# Autodesk Inventor assembly: ODrive Pro Assembly
(part 2 of 2)
- C:\work\openworkout\digital_weight_device\cad\v5\odrive\ODrive Pro Assembly\Leader_6_1.ipt
- C:\work\openworkout\digital_weight_device\cad\v5\odrive\ODrive Pro Assembly\Extruded_4_6.ipt
- C:\work\openworkout\digital_weight_device\cad\v5\odrive\ODrive Pro Assembly\Open CASCADE STEP translator 6.8 2.1.1_2_1.ipt
- C:\work\openworkout\digital_weight_device\cad\v5\odrive\ODrive Pro Assembly\Extruded_4_7.ipt
- C:\work\openworkout\digital_weight_device\cad\v5\odrive\ODrive Pro Assembly\Cylinder_6_2.ipt
- C:\work\openworkout\digital_weight_device\cad\v5\odrive\ODrive Pro Assembly\Lead_2.ipt
- C:\work\openworkout\digital_weight_device\cad\v5\odrive\ODrive Pro Assembly\RES 0603 (1608 metric)_8.ipt
- C:\work\openworkout\digital_weight_device\cad\v5\odrive\ODrive Pro Assembly\Open CASCADE STEP translator 6.8 1.2.1_2_1.ipt
- C:\work\openworkout\digital_weight_device\cad\v5\odrive\ODrive Pro Assembly\Extruded_21_4.ipt
- C:\work\openworkout\digital_weight_device\cad\v5\odrive\ODrive Pro Assembly\Extruded_58_1.ipt
- C:\work\openworkout\digital_weight_device\cad\v5\odrive\ODrive Pro Assembly\Extruded_64_1.ipt
- C:\work\openworkout\digital_weight_device\cad\v5\odrive\ODrive Pro Assembly\Extruded_38_1.ipt
- C:\work\openworkout\digital_weight_device\cad\v5\odrive\ODrive Pro Assembly\Extruded_39_3.ipt
- C:\work\openworkout\digital_weight_device\cad\v5\odrive\ODrive Pro Assembly\Thermal_Shape.ipt
- C:\work\openworkout\digital_weight_device\cad\v5\odrive\ODrive Pro Assembly\FDMS86300DC rev A.ipt
- C:\work\openworkout\digital_weight_device\cad\v5\odrive\ODrive Pro Assembly\________10 SIZE CODE G_7.ipt
- C:\work\openworkout\digital_weight_device\cad\v5\odrive\ODrive Pro Assembly\Extruded_27_1.ipt
- C:\work\openworkout\digital_weight_device\cad\v5\odrive\ODrive Pro Assembly\Extruded_28_5.ipt
- C:\work\openworkout\digital_weight_device\cad\v5\odrive\ODrive Pro Assembly\Mark_3_4.ipt
- C:\work\openworkout\digital_weight_device\cad\v5\odrive\ODrive Pro Assembly\Open CASCADE STEP translator 6.8 23.2.1_4_2.ipt
- C:\work\openworkout\digital_weight_device\cad\v5\odrive\ODrive Pro Assembly\Extruded_26_1.ipt
- C:\work\openworkout\digital_weight_device\cad\v5\odrive\ODrive Pro Assembly\Extruded_14_9.ipt
- C:\work\openworkout\digital_weight_device\cad\v5\odrive\ODrive Pro Assembly\______10 SIZE CODE G_1.ipt
- C:\work\openworkout\digital_weight_device\cad\v5\odrive\ODrive Pro Assembly\Leader_26.ipt
- C:\work\openworkout\digital_weight_device\cad\v5\odrive\ODrive Pro Assembly\Extruded_66.ipt
- C:\work\openworkout\digital_weight_device\cad\v5\odrive\ODrive Pro Assembly\Mark_1_4.ipt
- C:\work\openworkout\digital_weight_device\cad\v5\odrive\ODrive Pro Assembly\Mark_1_5.ipt
- C:\work\openworkout\digital_weight_device\cad\v5\odrive\ODrive Pro Assembly\Extruded_8_7.ipt
- C:\work\openworkout\digital_weight_device\cad\v5\odrive\ODrive Pro Assembly\Extruded_45_1.ipt
- C:\work\openworkout\digital_weight_device\cad\v5\odrive\ODrive Pro Assembly\Extruded_27_2.ipt
- C:\work\openworkout\digital_weight_device\cad\v5\odrive\ODrive Pro Assembly\Extruded_25_4.ipt
- C:\work\openworkout\digital_weight_device\cad\v5\odrive\ODrive Pro Assembly\FDMS86300DC rev A_11.ipt
- C:\work\openworkout\digital_weight_device\cad\v5\odrive\ODrive Pro Assembly\Extruded_16_5.ipt
- C:\work\openworkout\digital_weight_device\cad\v5\odrive\ODrive Pro Assembly\Extruded_51_1.ipt
- C:\work\openworkout\digital_weight_device\cad\v5\odrive\ODrive Pro Assembly\Open CASCADE STEP translator 6.8 23.2.1_7_1.ipt
- C:\work\openworkout\digital_weight_device\cad\v5\odrive\ODrive Pro Assembly\Open CASCADE STEP translator 6.8 1.2.1_5_1.ipt
- C:\work\openworkout\digital_weight_device\cad\v5\odrive\ODrive Pro Assembly\Cylinder_4_1.ipt
- C:\work\openworkout\digital_weight_device\cad\v5\odrive\ODrive Pro Assembly\Open CASCADE STEP translator 6.8 1.2.1_6.ipt
- C:\work\openworkout\digital_weight_device\cad\v5\odrive\ODrive Pro Assembly\RES 0603 (1608 metric)_19.ipt
- C:\work\openworkout\digital_weight_device\cad\v5\odrive\ODrive Pro Assembly\Extruded_5_10.ipt
- C:\work\openworkout\digital_weight_device\cad\v5\odrive\ODrive Pro Assembly\Extruded_21_5.ipt
- C:\work\openworkout\digital_weight_device\cad\v5\odrive\ODrive Pro Assembly\Mid_Body_6_1.ipt
- C:\work\openworkout\digital_weight_device\cad\v5\odrive\ODrive Pro Assembly\Extruded_23_4.ipt
- C:\work\openworkout\digital_weight_device\cad\v5\odrive\ODrive Pro Assembly\Cylinder_10_2.ipt
- C:\work\openworkout\digital_weight_device\cad\v5\odrive\ODrive Pro Assembly\Extruded_16_6.ipt
- C:\work\openworkout\digital_weight_device\cad\v5\odrive\ODrive Pro Assembly\Extruded_31_3.ipt
- C:\work\openworkout\digital_weight_device\cad\v5\odrive\ODrive Pro Assembly\Leader_4_2.ipt
- C:\work\openworkout\digital_weight_device\cad\v5\odrive\ODrive Pro Assembly\Leader_1_2.ipt
- C:\work\openworkout\digital_weight_device\cad\v5\odrive\ODrive Pro Assembly\Leader_12.ipt
- C:\work\openworkout\digital_weight_device\cad\v5\odrive\ODrive Pro Assembly\Leader_8.ipt
- C:\work\openworkout\digital_weight_device\cad\v5\odrive\ODrive Pro Assembly\Extruded_20_4.ipt
- C:\work\openworkout\digital_weight_device\cad\v5\odrive\ODrive Pro Assembly\Extruded_18_4.ipt
- C:\work\openworkout\digital_weight_device\cad\v5\odrive\ODrive Pro Assembly\RES 0603 (1608 metric)_4.ipt
- C:\work\openworkout\digital_weight_device\cad\v5\odrive\ODrive Pro Assembly\Open CASCADE STEP translator 6.8 2.1.1_7.ipt
- C:\work\openworkout\digital_weight_device\cad\v5\odrive\ODrive Pro Assembly\Extruded_4_8.ipt
- C:\work\openworkout\digital_weight_device\cad\v5\odrive\ODrive Pro Assembly\Extruded_8_8.ipt
- C:\work\openworkout\digital_weight_device\cad\v5\odrive\ODrive Pro Assembly\Cylinder_14.ipt
- C:\work\openworkout\digital_weight_device\cad\v5\odrive\ODrive Pro Assembly\Extruded_17_2.ipt
- C:\work\openworkout\digital_weight_device\cad\v5\odrive\ODrive Pro Assembly\Extruded_14_10.ipt
- C:\work\openworkout\digital_weight_device\cad\v5\odrive\ODrive Pro Assembly\Extruded_9_8.ipt
- C:\work\openworkout\digital_weight_device\cad\v5\odrive\ODrive Pro Assembly\Extruded_4_9.ipt
- C:\work\openworkout\digital_weight_device\cad\v5\odrive\ODrive Pro Assembly\Open CASCADE STEP translator 6.8 43.4.1_8.ipt
- C:\work\openworkout\digital_weight_device\cad\v5\odrive\ODrive Pro Assembly\Open CASCADE STEP translator 6.8 43.4.1_4.ipt
- C:\work\openworkout\digital_weight_device\cad\v5\odrive\ODrive Pro Assembly\Open CASCADE STEP translator 6.8 1.1.ipt
- C:\work\openworkout\digital_weight_device\cad\v5\odrive\ODrive Pro Assembly\Extruded_2_9.ipt
- C:\work\openworkout\digital_weight_device\cad\v5\odrive\ODrive Pro Assembly\Extruded_1_11.ipt
- C:\work\openworkout\digital_weight_device\cad\v5\odrive\ODrive Pro Assembly\Extruded_1_12.ipt
- C:\work\openworkout\digital_weight_device\cad\v5\odrive\ODrive Pro Assembly\Cylinder_10_3.ipt
- C:\work\openworkout\digital_weight_device\cad\v5\odrive\ODrive Pro Assembly\Extruded_3_11.ipt
- C:\work\openworkout\digital_weight_device\cad\v5\odrive\ODrive Pro Assembly\Extruded_1_13.ipt
- C:\work\openworkout\digital_weight_device\cad\v5\odrive\ODrive Pro Assembly\Open CASCADE STEP translator 6.8 2.2.1_3.ipt
- C:\work\openworkout\digital_weight_device\cad\v5\odrive\ODrive Pro Assembly\Open CASCADE STEP translator 6.8 19.1.2.ipt
- C:\work\openworkout\digital_weight_device\cad\v5\odrive\ODrive Pro Assembly\Extruded_2_10.ipt
- C:\work\openworkout\digital_weight_device\cad\v5\odrive\ODrive Pro Assembly\Extruded_67.ipt
- C:\work\openworkout\digital_weight_device\cad\v5\odrive\ODrive Pro Assembly\Extruded_21_6.ipt
- C:\work\openworkout\digital_weight_device\cad\v5\odrive\ODrive Pro Assembly\Extruded_15_8.ipt
- C:\work\openworkout\digital_weight_device\cad\v5\odrive\ODrive Pro Assembly\Leader_3_1.ipt
- C:\work\openworkout\digital_weight_device\cad\v5\odrive\ODrive Pro Assembly\Extruded_56_1.ipt
- C:\work\openworkout\digital_weight_device\cad\v5\odrive\ODrive Pro Assembly\Open CASCADE STEP translator 6.8 26.4.1_4.ipt
- C:\work\openworkout\digital_weight_device\cad\v5\odrive\ODrive Pro Assembly\Mark_9.ipt
- C:\work\openworkout\digital_weight_device\cad\v5\odrive\ODrive Pro Assembly\FDMS86300DC rev A_9.ipt
- C:\work\openworkout\digital_weight_device\cad\v5\odrive\ODrive Pro Assembly\FDMS86300DC rev A_5.ipt
- C:\work\openworkout\digital_weight_device\cad\v5\odrive\ODrive Pro Assembly\Extruded_45_2.ipt
- C:\work\openworkout\digital_weight_device\cad\v5\odrive\ODrive Pro Assembly\Open CASCADE STEP translator 6.8 1.2.1_3_1.ipt
- C:\work\openworkout\digital_weight_device\cad\v5\odrive\ODrive Pro Assembly\Open CASCADE STEP translator 6.8 1.2.1_1_1.ipt
- C:\work\openworkout\digital_weight_device\cad\v5\odrive\ODrive Pro Assembly\Extruded_27_3.ipt
- C:\work\openworkout\digital_weight_device\cad\v5\odrive\ODrive Pro Assembly\Extruded_30_4.ipt
- C:\work\openworkout\digital_weight_device\cad\v5\odrive\ODrive Pro Assembly\Open CASCADE STEP translator 6.8 23.2.1_14.ipt
- C:\work\openworkout\digital_weight_device\cad\v5\odrive\ODrive Pro Assembly\Extruded_17_3.ipt
- C:\work\openworkout\digital_weight_device\cad\v5\odrive\ODrive Pro Assembly\Extruded_16_7.ipt
- C:\work\openworkout\digital_weight_device\cad\v5\odrive\ODrive Pro Assembly\Cylinder_5_1.ipt
- C:\work\openworkout\digital_weight_device\cad\v5\odrive\ODrive Pro Assembly\Extruded_37_2.ipt
- C:\work\openworkout\digital_weight_device\cad\v5\odrive\ODrive Pro Assembly\Extruded_32_4.ipt
- C:\work\openworkout\digital_weight_device\cad\v5\odrive\ODrive Pro Assembly\Extruded_13_8.ipt
- C:\work\openworkout\digital_weight_device\cad\v5\odrive\ODrive Pro Assembly\Mark_2_4.ipt
- C:\work\openworkout\digital_weight_device\cad\v5\odrive\ODrive Pro Assembly\Extruded_18_5.ipt
- C:\work\openworkout\digital_weight_device\cad\v5\odrive\ODrive Pro Assembly\Extruded_38_2.ipt
- C:\work\openworkout\digital_weight_device\cad\v5\odrive\ODrive Pro Assembly\Extruded_11_7.ipt
- C:\work\openworkout\digital_weight_device\cad\v5\odrive\ODrive Pro Assembly\Extruded_4_10.ipt
- C:\work\openworkout\digital_weight_device\cad\v5\odrive\ODrive Pro Assembly\_______10x9.5L SIDE CODE G.ipt
- C:\work\openworkout\digital_weight_device\cad\v5\odrive\ODrive Pro Assembly\Extruded_17_4.ipt
- C:\work\openworkout\digital_weight_device\cad\v5\odrive\ODrive Pro Assembly\________10 SIZE CODE G_4.ipt
- C:\work\openworkout\digital_weight_device\cad\v5\odrive\ODrive Pro Assembly\_______10x9.5L SIDE CODE G_2.ipt
- C:\work\openworkout\digital_weight_device\cad\v5\odrive\ODrive Pro Assembly\Extruded_6_10.ipt
- C:\work\openworkout\digital_weight_device\cad\v5\odrive\ODrive Pro Assembly\Open CASCADE STEP translator 6.8 23.2.1_7_2.ipt
- C:\work\openworkout\digital_weight_device\cad\v5\odrive\ODrive Pro Assembly\Extruded_25_5.ipt
- C:\work\openworkout\digital_weight_device\cad\v5\odrive\ODrive Pro Assembly\Extruded_68.ipt
- C:\work\openworkout\digital_weight_device\cad\v5\odrive\ODrive Pro Assembly\LED 0603 APT1608 GREEN.ipt
- C:\work\openworkout\digital_weight_device\cad\v5\odrive\ODrive Pro Assembly\Extruded_2_11.ipt
- C:\work\openworkout\digital_weight_device\cad\v5\odrive\ODrive Pro Assembly\Mid_Body_10.ipt
- C:\work\openworkout\digital_weight_device\cad\v5\odrive\ODrive Pro Assembly\Mid_Body_1_4.ipt
- C:\work\openworkout\digital_weight_device\cad\v5\odrive\ODrive Pro Assembly\Extruded_5_11.ipt
- C:\work\openworkout\digital_weight_device\cad\v5\odrive\ODrive Pro Assembly\Extruded_20_5.ipt
- C:\work\openworkout\digital_weight_device\cad\v5\odrive\ODrive Pro Assembly\Cylinder_8_2.ipt
- C:\work\openworkout\digital_weight_device\cad\v5\odrive\ODrive Pro Assembly\Open CASCADE STEP translator 6.8 2.1.2_1_1.ipt
- C:\work\openworkout\digital_weight_device\cad\v5\odrive\ODrive Pro Assembly\Open CASCADE STEP translator 6.8 2.2.1_1_2.ipt
- C:\work\openworkout\digital_weight_device\cad\v5\odrive\ODrive Pro Assembly\Open CASCADE STEP translator 6.8 23.2.1_5_1.ipt
- C:\work\openworkout\digital_weight_device\cad\v5\odrive\ODrive Pro Assembly\Extruded_3_12.ipt
- C:\work\openworkout\digital_weight_device\cad\v5\odrive\ODrive Pro Assembly\RES 0603 (1608 metric)_10.ipt
- C:\work\openworkout\digital_weight_device\cad\v5\odrive\ODrive Pro Assembly\Extruded_1_14.ipt
- C:\work\openworkout\digital_weight_device\cad\v5\odrive\ODrive Pro Assembly\Extruded_13_9.ipt
- C:\work\openworkout\digital_weight_device\cad\v5\odrive\ODrive Pro Assembly\Thermal_Shape_1.ipt
- C:\work\openworkout\digital_weight_device\cad\v5\odrive\ODrive Pro Assembly\Leader_19.ipt
- C:\work\openworkout\digital_weight_device\cad\v5\odrive\ODrive Pro Assembly\Open CASCADE STEP translator 6.8 5.2.1_1.ipt
- C:\work\openworkout\digital_weight_device\cad\v5\odrive\ODrive Pro Assembly\Open CASCADE STEP translator 6.8 43.4.1_15.ipt
- C:\work\openworkout\digital_weight_device\cad\v5\odrive\ODrive Pro Assembly\Extruded_69.ipt
- C:\work\openworkout\digital_weight_device\cad\v5\odrive\ODrive Pro Assembly\Leader_31.ipt
- C:\work\openworkout\digital_weight_device\cad\v5\odrive\ODrive Pro Assembly\Leader_5_3.ipt
- C:\work\openworkout\digital_weight_device\cad\v5\odrive\ODrive Pro Assembly\Extruded_1_15.ipt
- C:\work\openworkout\digital_weight_device\cad\v5\odrive\ODrive Pro Assembly\Extruded_2_12.ipt
- C:\work\openworkout\digital_weight_device\cad\v5\odrive\ODrive Pro Assembly\Extruded_10_9.ipt
- C:\work\openworkout\digital_weight_device\cad\v5\odrive\ODrive Pro Assembly\Cylinder_5_2.ipt
- C:\work\openworkout\digital_weight_device\cad\v5\odrive\ODrive Pro Assembly\Lead_2_1.ipt
- C:\work\openworkout\digital_weight_device\cad\v5\odrive\ODrive Pro Assembly\Open CASCADE STEP translator 6.8 23.2.1_15.ipt
- C:\work\openworkout\digital_weight_device\cad\v5\odrive\ODrive Pro Assembly\Extruded_40_3.ipt
- C:\work\openworkout\digital_weight_device\cad\v5\odrive\ODrive Pro Assembly\RPC2512_stp_2.ipt
- C:\work\openworkout\digital_weight_device\cad\v5\odrive\ODrive Pro Assembly\Open CASCADE STEP translator 6.8 23.2.1_5_2.ipt
- C:\work\openworkout\digital_weight_device\cad\v5\odrive\ODrive Pro Assembly\Open CASCADE STEP translator 6.8 23.2.1_3_1.ipt
- C:\work\openworkout\digital_weight_device\cad\v5\odrive\ODrive Pro Assembly\Extruded_46_1.ipt
- C:\work\openworkout\digital_weight_device\cad\v5\odrive\ODrive Pro Assembly\Extruded_17_5.ipt
- C:\work\openworkout\digital_weight_device\cad\v5\odrive\ODrive Pro Assembly\Extruded_19_6.ipt
- C:\work\openworkout\digital_weight_device\cad\v5\odrive\ODrive Pro Assembly\Open CASCADE STEP translator 6.8 26.2.1.ipt
- C:\work\openworkout\digital_weight_device\cad\v5\odrive\ODrive Pro Assembly\Extruded_8_9.ipt
- C:\work\openworkout\digital_weight_device\cad\v5\odrive\ODrive Pro Assembly\________10 SIZE CODE G_6.ipt
- C:\work\openworkout\digital_weight_device\cad\v5\odrive\ODrive Pro Assembly\Extruded_26_2.ipt
- C:\work\openworkout\digital_weight_device\cad\v5\odrive\ODrive Pro Assembly\Extruded_27_4.ipt
- C:\work\openworkout\digital_weight_device\cad\v5\odrive\ODrive Pro Assembly\Open CASCADE STEP translator 6.8 23.2.1_7_3.ipt
- C:\work\openworkout\digital_weight_device\cad\v5\odrive\ODrive Pro Assembly\Mid_Body_2_4.ipt
- C:\work\openworkout\digital_weight_device\cad\v5\odrive\ODrive Pro Assembly\Extruded_53_1.ipt
- C:\work\openworkout\digital_weight_device\cad\v5\odrive\ODrive Pro Assembly\Extruded_1_16.ipt
- C:\work\openworkout\digital_weight_device\cad\v5\odrive\ODrive Pro Assembly\_______10x9.5L SIDE CODE G_1.ipt
- C:\work\openworkout\digital_weight_device\cad\v5\odrive\ODrive Pro Assembly\Leader_25.ipt
- C:\work\openworkout\digital_weight_device\cad\v5\odrive\ODrive Pro Assembly\Extruded_9_9.ipt
- C:\work\openworkout\digital_weight_device\cad\v5\odrive\ODrive Pro Assembly\Open CASCADE STEP translator 6.8 23.2.1_3_2.ipt
- C:\work\openworkout\digital_weight_device\cad\v5\odrive\ODrive Pro Assembly\Open CASCADE STEP translator 6.8 23.2.1_3_3.ipt
- C:\work\openworkout\digital_weight_device\cad\v5\odrive\ODrive Pro Assembly\Extruded_17_6.ipt
- C:\work\openworkout\digital_weight_device\cad\v5\odrive\ODrive Pro Assembly\Extruded_26_3.ipt
- C:\work\openworkout\digital_weight_device\cad\v5\odrive\ODrive Pro Assembly\Extruded_17_7.ipt
- C:\work\openworkout\digital_weight_device\cad\v5\odrive\ODrive Pro Assembly\Extruded_50_1.ipt
- C:\work\openworkout\digital_weight_device\cad\v5\odrive\ODrive Pro Assembly\Open CASCADE STEP translator 6.8 23.2.1_6_1.ipt
- C:\work\openworkout\digital_weight_device\cad\v5\odrive\ODrive Pro Assembly\Open CASCADE STEP translator 6.8 2.2.1_4.ipt
- C:\work\openworkout\digital_weight_device\cad\v5\odrive\ODrive Pro Assembly\Mid_Body_3_3.ipt
- C:\work\openworkout\digital_weight_device\cad\v5\odrive\ODrive Pro Assembly\Extruded_11_8.ipt
- C:\work\openworkout\digital_weight_device\cad\v5\odrive\ODrive Pro Assembly\Extruded_43_2.ipt
- C:\work\openworkout\digital_weight_device\cad\v5\odrive\ODrive Pro Assembly\Leader_2_2.ipt
- C:\work\openworkout\digital_weight_device\cad\v5\odrive\ODrive Pro Assembly\Open CASCADE STEP translator 6.8 26.4.1_7.ipt
- C:\work\openworkout\digital_weight_device\cad\v5\odrive\ODrive Pro Assembly\Open CASCADE STEP translator 6.8 18.2.1_1_2.ipt
- C:\work\openworkout\digital_weight_device\cad\v5\odrive\ODrive Pro Assembly\FDMS86300DC rev A_8.ipt
- C:\work\openworkout\digital_weight_device\cad\v5\odrive\ODrive Pro Assembly\Extruded_44_2.ipt
- C:\work\openworkout\digital_weight_device\cad\v5\odrive\ODrive Pro Assembly\Open CASCADE STEP translator 6.8 1.2.1_2_2.ipt
- C:\work\openworkout\digital_weight_device\cad\v5\odrive\ODrive Pro Assembly\Extruded_42_2.ipt
- C:\work\openworkout\digital_weight_device\cad\v5\odrive\ODrive Pro Assembly\Mark_5_1.ipt
- C:\work\openworkout\digital_weight_device\cad\v5\odrive\ODrive Pro Assembly\Mid_Body_1_5.ipt
- C:\work\openworkout\digital_weight_device\cad\v5\odrive\ODrive Pro Assembly\Extruded_20_6.ipt
- C:\work\openworkout\digital_weight_device\cad\v5\odrive\ODrive Pro Assembly\Extruded_15_9.ipt
- C:\work\openworkout\digital_weight_device\cad\v5\odrive\ODrive Pro Assembly\Extruded_31_4.ipt
- C:\work\openworkout\digital_weight_device\cad\v5\odrive\ODrive Pro Assembly\RES 0603 (1608 metric)_3.ipt
- C:\work\openworkout\digital_weight_device\cad\v5\odrive\ODrive Pro Assembly\Cylinder_12_1.ipt
- C:\work\openworkout\digital_weight_device\cad\v5\odrive\ODrive Pro Assembly\Cylinder_17.ipt
- C:\work\openworkout\digital_weight_device\cad\v5\odrive\ODrive Pro Assembly\Extruded_16_8.ipt
- C:\work\openworkout\digital_weight_device\cad\v5\odrive\ODrive Pro Assembly\Extruded_8_10.ipt
- C:\work\openworkout\digital_weight_device\cad\v5\odrive\ODrive Pro Assembly\Open CASCADE STEP translator 6.8 43.4.1_7.ipt
- C:\work\openworkout\digital_weight_device\cad\v5\odrive\ODrive Pro Assembly\Cylinder_19.ipt
- C:\work\openworkout\digital_weight_device\cad\v5\odrive\ODrive Pro Assembly\Extruded_6_11.ipt
- C:\work\openworkout\digital_weight_device\cad\v5\odrive\ODrive Pro Assembly\Cylinder_9_2.ipt
- C:\work\openworkout\digital_weight_device\cad\v5\odrive\ODrive Pro Assembly\Extruded_2_13.ipt
- C:\work\openworkout\digital_weight_device\cad\v5\odrive\ODrive Pro Assembly\Open CASCADE STEP translator 6.8 2.1.2_4.ipt
- C:\work\openworkout\digital_weight_device\cad\v5\odrive\ODrive Pro Assembly\Extruded_4_11.ipt
- C:\work\openworkout\digital_weight_device\cad\v5\odrive\ODrive Pro Assembly\Extruded_26_4.ipt
- C:\work\openworkout\digital_weight_device\cad\v5\odrive\ODrive Pro Assembly\Mid_Body_11.ipt
- C:\work\openworkout\digital_weight_device\cad\v5\odrive\ODrive Pro Assembly\Extruded_35_3.ipt
- C:\work\openworkout\digital_weight_device\cad\v5\odrive\ODrive Pro Assembly\Cylinder_4_2.ipt
- C:\work\openworkout\digital_weight_device\cad\v5\odrive\ODrive Pro Assembly\Extruded_36_2.ipt
- C:\work\openworkout\digital_weight_device\cad\v5\odrive\ODrive Pro Assembly\Extruded_27_5.ipt
- C:\work\openworkout\digital_weight_device\cad\v5\odrive\ODrive Pro Assembly\Open CASCADE STEP translator 6.8 23.2.1_5_3.ipt
- C:\work\openworkout\digital_weight_device\cad\v5\odrive\ODrive Pro Assembly\Extruded_18_6.ipt
- C:\work\openworkout\digital_weight_device\cad\v5\odrive\ODrive Pro Assembly\Extruded_5_12.ipt
- C:\work\openworkout\digital_weight_device\cad\v5\odrive\ODrive Pro Assembly\lead_1_1.ipt
- C:\work\openworkout\digital_weight_device\cad\v5\odrive\ODrive Pro Assembly\___________10 SIZE CODE G_5.ipt
- C:\work\openworkout\digital_weight_device\cad\v5\odrive\ODrive Pro Assembly\Extruded_3_13.ipt
- C:\work\openworkout\digital_weight_device\cad\v5\odrive\ODrive Pro Assembly\Open CASCADE STEP translator 6.8 23.2.1_6_2.ipt
- C:\work\openworkout\digital_weight_device\cad\v5\odrive\ODrive Pro Assembly\Extruded_11_9.ipt
- C:\work\openworkout\digital_weight_device\cad\v5\odrive\ODrive Pro Assembly\Open CASCADE STEP translator 6.8 2.4.1.ipt
- C:\work\openworkout\digital_weight_device\cad\v5\odrive\ODrive Pro Assembly\Mark_1_6.ipt
- C:\work\openworkout\digital_weight_device\cad\v5\odrive\ODrive Pro Assembly\Extruded_4_12.ipt
- C:\work\openworkout\digital_weight_device\cad\v5\odrive\ODrive Pro Assembly\�г�-����2.ipt
- C:\work\openworkout\digital_weight_device\cad\v5\odrive\ODrive Pro Assembly\Open CASCADE STEP translator 6.8 2.1.1_1_2.ipt
- C:\work\openworkout\digital_weight_device\cad\v5\odrive\ODrive Pro Assembly\Open CASCADE STEP translator 6.8 2.1.2_1_2.ipt
- C:\work\openworkout\digital_weight_device\cad\v5\odrive\ODrive Pro Assembly\Extruded_7_10.ipt
- C:\work\openworkout\digital_weight_device\cad\v5\odrive\ODrive Pro Assembly\RES 0603 (1608 metric)_9.ipt
- C:\work\openworkout\digital_weight_device\cad\v5\odrive\ODrive Pro Assembly\Extruded_70.ipt
- C:\work\openworkout\digital_weight_device\cad\v5\odrive\ODrive Pro Assembly\Extruded_12_10.ipt
- C:\work\openworkout\digital_weight_device\cad\v5\odrive\ODrive Pro Assembly\Open CASCADE STEP translator 6.8 43.2.1.ipt
- C:\work\openworkout\digital_weight_device\cad\v5\odrive\ODrive Pro Assembly\Leader_18.ipt
- C:\work\openworkout\digital_weight_device\cad\v5\odrive\ODrive Pro Assembly\Open CASCADE STEP translator 6.8 43.4.1_14.ipt
- C:\work\openworkout\digital_weight_device\cad\v5\odrive\ODrive Pro Assembly\Extruded_17_8.ipt
- C:\work\openworkout\digital_weight_device\cad\v5\odrive\ODrive Pro Assembly\Leader_4_3.ipt
- C:\work\openworkout\digital_weight_device\cad\v5\odrive\ODrive Pro Assembly\Extruded_3_14.ipt
- C:\work\openworkout\digital_weight_device\cad\v5\odrive\ODrive Pro Assembly\Extruded_71.ipt
- C:\work\openworkout\digital_weight_device\cad\v5\odrive\ODrive Pro Assembly\Lead_5.ipt
- C:\work\openworkout\digital_weight_device\cad\v5\odrive\ODrive Pro Assembly\RPC2512_stp_3.ipt
- C:\work\openworkout\digital_weight_device\cad\v5\odrive\ODrive Pro Assembly\Open CASCADE STEP translator 6.8 23.2.1_4_3.ipt
- C:\work\openworkout\digital_weight_device\cad\v5\odrive\ODrive Pro Assembly\Extruded_7_11.ipt
- C:\work\openworkout\digital_weight_device\cad\v5\odrive\ODrive Pro Assembly\Extruded_22_5.ipt
- C:\work\openworkout\digital_weight_device\cad\v5\odrive\ODrive Pro Assembly\Extruded_33_3.ipt
- C:\work\openworkout\digital_weight_device\cad\v5\odrive\ODrive Pro Assembly\Leader_3_2.ipt
- C:\work\openworkout\digital_weight_device\cad\v5\odrive\ODrive Pro Assembly\Leader_11.ipt
- C:\work\openworkout\digital_weight_device\cad\v5\odrive\ODrive Pro Assembly\ODrive Pro Enclosure Top.ipt
- C:\work\openworkout\digital_weight_device\cad\v5\odrive\ODrive Pro Assembly\ODrive Pro Enclosure Base Plate.ipt
- C:\work\openworkout\digital_weight_device\cad\v5\odrive\ODrive Pro Assembly\Thermal Pad ODrive Pro.ipt
- C:\work\openworkout\digital_weight_device\cad\v5\odrive\ODrive Pro Assembly\90991A112_18-8 Stainless Steel Button Head Torx Screws.ipt
## Components (728 placed, 728 different names)
1. NAUO1
2. NAUO2
3. NAUO3
4. NAUO4
5. NAUO5
6. NAUO6
7. NAUO7
8. NAUO8
9. NAUO9
10. NAUO10
11. NAUO11
12. NAUO12
13. NAUO13
14. NAUO14
15. NAUO15
16. NAUO16
17. NAUO17
18. NAUO18
19. NAUO19
20. NAUO20
21. NAUO21
22. NAUO22
23. NAUO23
24. NAUO24
25. NAUO25
26. NAUO26
27. NAUO27
28. NAUO28
29. NAUO29
30. NAUO30
31. NAUO31
32. NAUO32
33. NAUO33
34. NAUO34
35. NAUO35
36. NAUO36
37. NAUO37
38. NAUO38
39. NAUO39
40. NAUO40
41. NAUO41
42. NAUO42
43. NAUO43
44. NAUO44
45. NAUO45
46. NAUO46
47. NAUO47
48. NAUO48
49. NAUO49
50. NAUO50
51. NAUO51
52. NAUO52
53. NAUO53
54. NAUO54
55. NAUO55
56. NAUO56
57. NAUO57
58. NAUO58
59. NAUO59
60. NAUO60
61. NAUO61
62. NAUO62
63. NAUO63
64. NAUO64
65. NAUO65
66. NAUO66
67. NAUO67
68. NAUO68
69. NAUO69
70. NAUO70
71. NAUO71
72. NAUO72
73. NAUO73
74. NAUO74
75. NAUO75
76. NAUO76
77. NAUO77
78. NAUO78
79. NAUO79
80. NAUO80
81. NAUO81
82. NAUO82
83. NAUO83
84. NAUO84
85. NAUO85
86. NAUO86
87. NAUO87
88. NAUO88
89. NAUO89
90. NAUO90
91. NAUO91
92. NAUO92
93. NAUO93
94. NAUO94
95. NAUO95
96. NAUO96
97. NAUO97
98. NAUO98
99. NAUO99
100. NAUO100
101. NAUO101
102. NAUO102
103. NAUO103
104. NAUO104
105. NAUO105
106. NAUO106
107. NAUO107
108. NAUO108
109. NAUO109
110. NAUO110
111. NAUO111
112. NAUO112
113. NAUO113
114. NAUO114
115. NAUO115
116. NAUO116
117. NAUO117
118. NAUO118
119. NAUO119
120. NAUO120
121. NAUO121
122. NAUO122
123. NAUO123
124. NAUO124
125. NAUO125
126. NAUO126
127. NAUO127
128. NAUO128
129. NAUO129
130. NAUO130
131. NAUO131
132. NAUO132
133. NAUO133
134. NAUO134
135. NAUO135
136. NAUO136
137. NAUO137
138. NAUO138
139. NAUO139
140. NAUO140
141. NAUO141
142. NAUO142
143. NAUO143
144. NAUO144
145. NAUO145
146. NAUO146
147. NAUO147
148. NAUO148
149. NAUO149
150. NAUO150
151. NAUO151
152. NAUO152
153. NAUO153
154. NAUO154
155. NAUO155
156. NAUO156
157. NAUO157
158. NAUO158
159. NAUO159
160. NAUO160
161. NAUO161
162. NAUO162
163. NAUO163
164. NAUO164
165. NAUO165
166. NAUO166
167. NAUO167
168. NAUO168
169. NAUO169
170. NAUO170
171. NAUO171
172. NAUO172
173. NAUO173
174. NAUO174
175. NAUO175
176. NAUO176
177. NAUO177
178. NAUO178
179. NAUO179
180. NAUO180
181. NAUO181
182. NAUO182
183. NAUO183
184. NAUO184
185. NAUO185
186. NAUO186
187. NAUO187
188. NAUO188
189. NAUO189
190. NAUO190
191. NAUO191
192. NAUO192
193. NAUO193
194. NAUO194
195. NAUO195
196. NAUO196
197. NAUO197
198. NAUO198
199. NAUO199
200. NAUO200
201. NAUO201
202. NAUO202
203. NAUO203
204. NAUO204
205. NAUO205
206. NAUO206
207. NAUO207
208. NAUO208
209. NAUO209
210. NAUO210
211. NAUO211
212. NAUO212
213. NAUO213
214. NAUO214
215. NAUO215
216. NAUO216
217. NAUO217
218. NAUO218
219. NAUO219
220. NAUO220
221. NAUO221
222. NAUO222
223. NAUO223
224. NAUO224
225. NAUO225
226. NAUO226
227. NAUO227
228. NAUO228
229. NAUO229
230. NAUO230
231. NAUO231
232. NAUO232
233. NAUO233
234. NAUO234
235. NAUO235
236. NAUO236
237. NAUO237
238. NAUO238
239. NAUO239
240. NAUO240
241. NAUO241
242. NAUO242
243. NAUO243
244. NAUO244
245. NAUO245
246. NAUO246
247. NAUO247
248. NAUO248
249. NAUO249
250. NAUO250
251. NAUO251
252. NAUO252
253. NAUO253
254. NAUO254
255. NAUO255
256. NAUO256
257. NAUO257
258. NAUO258
259. NAUO259
260. NAUO260
261. NAUO261
262. NAUO262
263. NAUO263
264. NAUO264
265. NAUO265
266. NAUO266
267. NAUO267
268. NAUO268
269. NAUO269
270. NAUO270
271. NAUO271
272. NAUO272
273. NAUO273
274. NAUO274
275. NAUO275
276. NAUO276
277. NAUO277
278. NAUO278
279. NAUO279
280. NAUO280
281. NAUO281
282. NAUO282
283. NAUO283
284. NAUO284
285. NAUO285
286. NAUO286
287. NAUO287
288. NAUO288
289. NAUO289
290. NAUO290
291. NAUO291
292. NAUO292
293. NAUO293
294. NAUO294
295. NAUO295
296. NAUO296
297. NAUO297
298. NAUO298
299. NAUO299
300. NAUO300
301. NAUO301
302. NAUO302
303. NAUO303
304. NAUO304
305. NAUO305
306. NAUO306
307. NAUO307
308. NAUO308
309. NAUO309
310. NAUO310
311. NAUO311
312. NAUO312
313. NAUO313
314. NAUO314
315. NAUO315
316. NAUO316
317. NAUO317
318. NAUO318
319. NAUO319
320. NAUO320
321. NAUO321
322. NAUO322
323. NAUO323
324. NAUO324
325. NAUO325
326. NAUO326
327. NAUO327
328. NAUO328
329. NAUO329
330. NAUO330
331. NAUO331
332. NAUO332
333. NAUO333
334. NAUO334
335. NAUO335
336. NAUO336
337. NAUO337
338. NAUO338
339. NAUO339
340. NAUO340
341. NAUO341
342. NAUO342
343. NAUO343
344. NAUO344
345. NAUO345
346. NAUO346
347. NAUO347
348. NAUO348
349. NAUO349
350. NAUO350
351. NAUO351
352. NAUO352
353. NAUO353
354. NAUO354
355. NAUO355
356. NAUO356
357. NAUO357
358. NAUO358
359. NAUO359
360. NAUO360
361. NAUO361
362. NAUO362
363. NAUO363
364. NAUO364
365. NAUO365
366. NAUO366
367. NAUO367
368. NAUO368
369. NAUO369
370. NAUO370
371. NAUO371
372. NAUO372
373. NAUO373
374. NAUO374
375. NAUO375
376. NAUO376
377. NAUO377
378. NAUO378
379. NAUO379
380. NAUO380
381. NAUO381
382. NAUO382
383. NAUO383
384. NAUO384
385. NAUO385
386. NAUO386
387. NAUO387
388. NAUO388
389. NAUO389
390. NAUO390
391. NAUO391
392. NAUO392
393. NAUO393
394. NAUO394
395. NAUO395
396. NAUO396
397. NAUO397
398. NAUO398
399. NAUO399
400. NAUO400
401. NAUO401
402. NAUO402
403. NAUO403
404. NAUO404
405. NAUO405
406. NAUO406
407. NAUO407
408. NAUO408
409. NAUO409
410. NAUO410
411. NAUO411
412. NAUO412
413. NAUO413
414. NAUO414
415. NAUO415
416. NAUO416
417. NAUO417
418. NAUO418
419. NAUO419
420. NAUO420
421. NAUO421
422. NAUO422
423. NAUO423
424. NAUO424
425. NAUO425
426. NAUO426
427. NAUO427
428. NAUO428
429. NAUO429
430. NAUO430
431. NAUO431
432. NAUO432
433. NAUO433
434. NAUO434
435. NAUO435
436. NAUO436
437. NAUO437
438. NAUO438
439. NAUO439
440. NAUO440
441. NAUO441
442. NAUO442
443. NAUO443
444. NAUO444
445. NAUO445
446. NAUO446
447. NAUO447
448. NAUO448
449. NAUO449
450. NAUO450
451. NAUO451
452. NAUO452
453. NAUO453
454. NAUO454
455. NAUO455
456. NAUO456
457. NAUO457
458. NAUO458
459. NAUO459
460. NAUO460
461. NAUO461
462. NAUO462
463. NAUO463
464. NAUO464
465. NAUO465
466. NAUO466
467. NAUO467
468. NAUO468
469. NAUO469
470. NAUO470
471. NAUO471
472. NAUO472
473. NAUO473
474. NAUO474
475. NAUO475
476. NAUO476
477. NAUO477
478. NAUO478
479. NAUO479
480. NAUO480
481. NAUO481
482. NAUO482
483. NAUO483
484. NAUO484
485. NAUO485
486. NAUO486
487. NAUO487
488. NAUO488
489. NAUO489
490. NAUO490
491. NAUO491
492. NAUO492
493. NAUO493
494. NAUO494
495. NAUO495
496. NAUO496
497. NAUO497
498. NAUO498
499. NAUO499
500. NAUO500
501. NAUO501
502. NAUO502
503. NAUO503
504. NAUO504
505. NAUO505
506. NAUO506
507. NAUO507
508. NAUO508
509. NAUO509
510. NAUO510
511. NAUO511
512. NAUO512
513. NAUO513
514. NAUO514
515. NAUO515
516. NAUO516
517. NAUO517
518. NAUO518
519. NAUO519
520. NAUO520
521. NAUO521
522. NAUO522
523. NAUO523
524. NAUO524
525. NAUO525
526. NAUO526
527. NAUO527
528. NAUO528
529. NAUO529
530. NAUO530
531. NAUO531
532. NAUO532
533. NAUO533
534. NAUO534
535. NAUO535
536. NAUO536
537. NAUO537
538. NAUO538
539. NAUO539
540. NAUO540
541. NAUO541
542. NAUO542
543. NAUO543
544. NAUO544
545. NAUO545
546. NAUO546
547. NAUO547
548. NAUO548
549. NAUO549
550. NAUO550
551. NAUO551
552. NAUO552
553. NAUO553
554. NAUO554
555. NAUO555
556. NAUO556
557. NAUO557
558. NAUO558
559. NAUO559
560. NAUO560
561. NAUO561
562. NAUO562
563. NAUO563
564. NAUO564
565. NAUO565
566. NAUO566
567. NAUO567
568. NAUO568
569. NAUO569
570. NAUO570
571. NAUO571
572. NAUO572
573. NAUO573
574. NAUO574
575. NAUO575
576. NAUO576
577. NAUO577
578. NAUO578
579. NAUO579
580. NAUO580
581. NAUO581
582. NAUO582
583. NAUO583
584. NAUO584
585. NAUO585
586. NAUO586
587. NAUO587
588. NAUO588
589. NAUO589
590. NAUO590
591. NAUO591
592. NAUO592
593. NAUO593
594. NAUO594
595. NAUO595
596. NAUO596
597. NAUO597
598. NAUO598
599. NAUO599
600. NAUO600
601. NAUO601
602. NAUO602
603. NAUO603
604. NAUO604
605. NAUO605
606. NAUO606
607. NAUO607
608. NAUO608
609. NAUO609
610. NAUO610
611. NAUO611
612. NAUO612
613. NAUO613
614. NAUO614
615. NAUO615
616. NAUO616
617. NAUO617
618. NAUO618
619. NAUO619
620. NAUO620
621. NAUO621
622. NAUO622
623. NAUO623
624. NAUO624
625. NAUO625
626. NAUO626
627. NAUO627
628. NAUO628
629. NAUO629
630. NAUO630
631. NAUO631
632. NAUO632
633. NAUO633
634. NAUO634
635. NAUO635
636. NAUO636
637. NAUO637
638. NAUO638
639. NAUO639
640. NAUO640
641. NAUO641
642. NAUO642
643. NAUO643
644. NAUO644
645. NAUO645
646. NAUO646
647. NAUO647
648. NAUO648
649. NAUO649
650. NAUO650
651. NAUO651
652. NAUO652
653. NAUO653
654. NAUO654
655. NAUO655
656. NAUO656
657. NAUO657
658. NAUO658
659. NAUO659
660. NAUO660
661. NAUO661
662. NAUO662
663. NAUO663
664. NAUO664
665. NAUO665
666. NAUO666
667. NAUO667
668. NAUO668
669. NAUO669
670. NAUO670
671. NAUO671
672. NAUO672
673. NAUO673
674. NAUO674
675. NAUO675
676. NAUO676
677. NAUO677
678. NAUO678
679. NAUO679
680. NAUO680
681. NAUO681
682. NAUO682
683. NAUO683
684. NAUO684
685. NAUO685
686. NAUO686
687. NAUO687
688. NAUO688
689. NAUO689
690. NAUO690
691. NAUO691
692. NAUO692
693. NAUO693
694. NAUO694
695. NAUO695
696. NAUO696
697. NAUO697
698. NAUO698
699. NAUO699
700. NAUO700
701. NAUO701
702. NAUO702
703. NAUO703
704. NAUO704
705. NAUO705
706. NAUO706
707. NAUO707
708. NAUO708
709. NAUO709
710. NAUO710
711. NAUO711
712. NAUO712
713. NAUO713
714. NAUO714
715. NAUO715
716. NAUO716
717. NAUO717
718. NAUO718
719. NAUO719
720. NAUO720
721. NAUO721
722. NAUO722
723. NAUO723
724. NAUO724
725. NAUO725
726. NAUO726
727. NAUO727
728. NAUO728
